# Autodesk Inventor assembly: Ensamblaje1
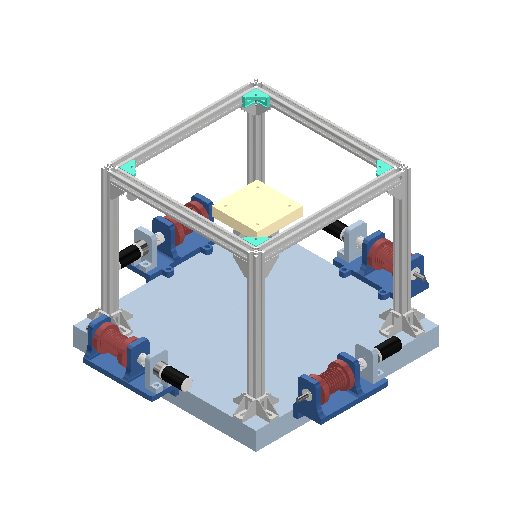
[picture p0: Inventor's stored thumbnail of the model, 512x512]
Saved by Autodesk Inventor 2026.1 (Build 301233000, 233)
## iProperties
Created: 2025-06-30
Part Number: Ensamblaje1
Document SubType Name: Assembly
Designer: piero
Author: piero
## Documents named in this file (10)
- D:\Tesis\Modelo 3D\CAD\Ensamblaje1.iam
- D:\Tesis\Modelo 3D\CAD\V-slot.ipt
- D:\Tesis\Modelo 3D\CAD\Plataforma.ipt
- D:\Tesis\Modelo 3D\CAD\Esquinero.ipt
- D:\Tesis\Modelo 3D\CAD\V-slot_2.ipt
- D:\Tesis\Modelo 3D\CAD\Soporte gancho.ipt
- D:\Tesis\Modelo 3D\CAD\Gancho.ipt
- D:\Tesis\Modelo 3D\CAD\Ensamblaje - 2.iam
- D:\Tesis\Modelo 3D\CAD\Mesa.ipt
- D:\Tesis\Modelo 3D\CAD\Polea\Polea.ipt
## Components (47 placed, 9 different names)
1. Mesa:1 — Coincidencia:10, Coincidencia:15, Coincidencia:22, Coincidencia:26, Nivelación:17, Nivelación:18, Coincidencia:30, Coincidencia:31, Coincidencia:32, Coincidencia:33, Coincidencia:36, Coincidencia:37, Coincidencia:38, Coincidencia:39, Coincidencia:44
2. V-slot:1 — Coincidencia:3, Nivelación:5, Nivelación:6, Nivelación:7, Nivelación:8, Coincidencia:4, Coincidencia:11, Nivelación:13, Nivelación:14, Coincidencia:14, Coincidencia:25, Nivelación:15, Nivelación:16
3. V-slot:2 — Nivelación:9, Nivelación:10, Coincidencia:5, Coincidencia:6, Nivelación:11, Nivelación:12
4. V-slot:3 — Coincidencia:7, Coincidencia:8, Coincidencia:9
5. V-slot:4 — Nivelación:1, Nivelación:2, Coincidencia:1, Nivelación:3, Nivelación:4, Coincidencia:2, Coincidencia:10, Nivelación:17, Nivelación:18
6. Plataforma:1
7. V-slot_2:1 — Nivelación:7, Nivelación:8, Coincidencia:4, Nivelación:9, Nivelación:10, Coincidencia:5, Coincidencia:13, Coincidencia:28
8. V-slot_2:2 — Nivelación:1, Nivelación:2, Coincidencia:1, Coincidencia:8, Coincidencia:9
9. V-slot_2:3 — Coincidencia:6, Nivelación:11, Nivelación:12, Coincidencia:7
10. V-slot_2:4 — Nivelación:3, Nivelación:4, Coincidencia:2, Coincidencia:3, Nivelación:5, Nivelación:6, Coincidencia:12, Coincidencia:27
11. Polea:1
12. Esquinero:6 — Coincidencia:13, Nivelación:14, Coincidencia:14
13. Esquinero:5 — Coincidencia:11, Nivelación:13, Coincidencia:12
14. Ensamblaje - 2:1 [sub-assembly] — Coincidencia:22, Coincidencia:44
15. Soporte gancho:1 — Nivelación:16, Coincidencia:27, Coincidencia:28, Coincidencia:29
16. Gancho:1 — Coincidencia:29
17. Esquinero:11
18. Esquinero:12
19. Ensamblaje - 2:2 [sub-assembly]
20. Soporte gancho:2
21. Gancho:2
22. Esquinero:17
23. Esquinero:18
24. Ensamblaje - 2:3 [sub-assembly]
25. Soporte gancho:3
26. Gancho:3
27. Esquinero:23
28. Esquinero:24
29. Ensamblaje - 2:4 [sub-assembly]
30. Soporte gancho:4
31. Gancho:4
32. Esquinero:7 — Coincidencia:25, Nivelación:15, Coincidencia:26
33. Esquinero:8
34. Esquinero:9
35. Esquinero:10
36. Esquinero:13
37. Esquinero:14
38. Esquinero:15
39. Esquinero:16
40. Esquinero:19
41. Esquinero:20
42. Esquinero:21
43. Esquinero:22
44. Esquinero:25
45. Esquinero:26
46. Esquinero:27
47. Esquinero:28
## Component patterns: (4 elements, first: Esquinero:6 + Esquinero:5 + Ensamblaje - 2:1 + Soporte gancho:1 + Gancho:1), (4 elements, first: Esquinero:7), Patrón de componentes 2:2 (4 elements), Patrón de componentes 2:3 (4 elements), Patrón de componentes 2:4 (4 elements)
## Relationships (54: Mate 36, Flush 18)
- Nivelación:1 [Flush]: V-slot:4 ↔ V-slot_2:2
- Nivelación:2 [Flush]: V-slot:4 ↔ V-slot_2:2
- Coincidencia:1 [Mate]: V-slot:4 ↔ V-slot_2:2
- Nivelación:3 [Flush]: V-slot:4 ↔ V-slot_2:4
- Nivelación:4 [Flush]: V-slot:4 ↔ V-slot_2:4
- Coincidencia:2 [Mate]: V-slot:4 ↔ V-slot_2:4
- Coincidencia:3 [Mate]: V-slot:1 ↔ V-slot_2:4
- Nivelación:5 [Flush]: V-slot:1 ↔ V-slot_2:4
- Nivelación:6 [Flush]: V-slot:1 ↔ V-slot_2:4
- Nivelación:7 [Flush]: V-slot:1 ↔ V-slot_2:1
- Nivelación:8 [Flush]: V-slot:1 ↔ V-slot_2:1
- Coincidencia:4 [Mate]: V-slot:1 ↔ V-slot_2:1
- Nivelación:9 [Flush]: V-slot:2 ↔ V-slot_2:1
- Nivelación:10 [Flush]: V-slot:2 ↔ V-slot_2:1
- Coincidencia:5 [Mate]: V-slot:2 ↔ V-slot_2:1
- Coincidencia:6 [Mate]: V-slot:2 ↔ V-slot_2:3
- Nivelación:11 [Flush]: V-slot:2 ↔ V-slot_2:3
- Nivelación:12 [Flush]: V-slot:2 ↔ V-slot_2:3
- Coincidencia:7 [Mate]: V-slot:3 ↔ V-slot_2:3
- Coincidencia:8 [Mate]: V-slot:3 ↔ V-slot_2:2
- Coincidencia:9 [Mate]: V-slot:3 ↔ V-slot_2:2
- Coincidencia:10 [Mate]: Mesa:1 ↔ V-slot:4
- Coincidencia:11 [Mate]: V-slot:1 ↔ Esquinero:5
- Nivelación:13 [Flush]: V-slot:1 ↔ Esquinero:5
- Coincidencia:12 [Mate]: V-slot_2:4 ↔ Esquinero:5
- Coincidencia:13 [Mate]: V-slot_2:1 ↔ Esquinero:6
- Nivelación:14 [Flush]: V-slot:1 ↔ Esquinero:6
- Coincidencia:14 [Mate]: V-slot:1 ↔ Esquinero:6
- Coincidencia:15 [Mate]: Mesa:1
- Coincidencia:22 [Mate]: Mesa:1 ↔ Ensamblaje - 2:1
- Coincidencia:25 [Mate]: V-slot:1 ↔ Esquinero:7
- Nivelación:15 [Flush]: V-slot:1 ↔ Esquinero:7
- Coincidencia:26 [Mate]: Mesa:1 ↔ Esquinero:7
- Nivelación:16 [Flush]: V-slot:1 ↔ Soporte gancho:1
- Coincidencia:27 [Mate]: V-slot_2:4 ↔ Soporte gancho:1
- Coincidencia:28 [Mate]: V-slot_2:1 ↔ Soporte gancho:1
- Coincidencia:29 [Mate]: Soporte gancho:1 ↔ Gancho:1
- Nivelación:17 [Flush] (30 mm): Mesa:1 ↔ V-slot:4
- Nivelación:18 [Flush] (30 mm): Mesa:1 ↔ V-slot:4
- Coincidencia:30 [Mate]: Mesa:1
- Coincidencia:31 [Mate]: Mesa:1
- Coincidencia:32 [Mate]: Mesa:1
- Coincidencia:33 [Mate]: Mesa:1
- Coincidencia:34 [Mate]
- Coincidencia:35 [Mate]
- Coincidencia:36 [Mate]: Mesa:1
- Coincidencia:37 [Mate]: Mesa:1
- Coincidencia:38 [Mate]: Mesa:1
- Coincidencia:39 [Mate]: Mesa:1
- Coincidencia:40 [Mate]
- Coincidencia:41 [Mate]
- Coincidencia:42 [Mate]
- Coincidencia:43 [Mate]
- Coincidencia:44 [Mate]: Mesa:1 ↔ Ensamblaje - 2:1
